# Autodesk Inventor assembly: Separator
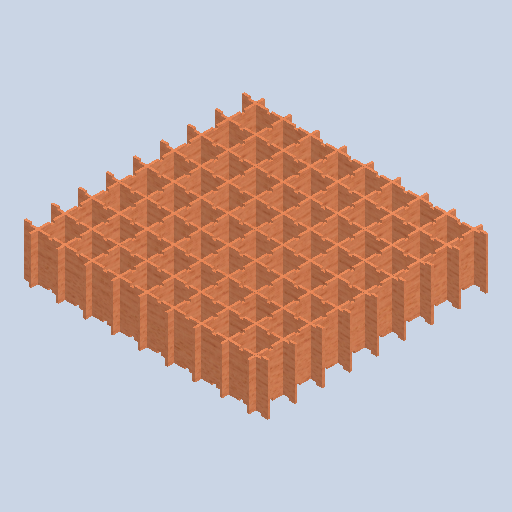
[picture p0: Inventor's stored thumbnail of the model, 512x512]
Saved by Autodesk Inventor 2024 (Build 280153000, 153)
## iProperties
Created: 2023-07-19
Part Number: Separator
Document SubType Name: Assembly
Designer: Bruno
Author: Bruno
## Documents named in this file (3)
- C:\Users\Bruno\brucloud\utn\td2\proyecto\autodesk\SeparatorAssembly.iam
- C:\Users\Bruno\brucloud\utn\td2\proyecto\autodesk\SeparatorPiece.ipt
- C:\Users\Bruno\brucloud\utn\td2\proyecto\autodesk\SeparatorPiece2.ipt
## Components (18 placed, 3 different names)
1. Separator — Rigid:3
2. SeparatorPiece:2
3. SeparatorPiece:3
4. SeparatorPiece:4
5. SeparatorPiece:5
6. SeparatorPiece:6
7. SeparatorPiece:7
8. SeparatorPiece:8
9. SeparatorPiece:9
10. SeparatorPiece2:1 — Rigid:3
11. SeparatorPiece2:2
12. SeparatorPiece2:3
13. SeparatorPiece2:4
14. SeparatorPiece2:5
15. SeparatorPiece2:6
16. SeparatorPiece2:7
17. SeparatorPiece2:8
18. SeparatorPiece2:9
## Component patterns: (9 elements, first: Separator), (9 elements, first: SeparatorPiece2:1)
## Relationships (1: WeldJoint 1)
- Rigid:3 [WeldJoint]: Separator ↔ SeparatorPiece2:1
## Named parameters: d0_d6 = 50.8 mm, d1_d7 = 35 mm, d2_d8 = 1, d4_d9 = 9, d8_d3 = 1
